# Autodesk Inventor assembly: assembly_hoop
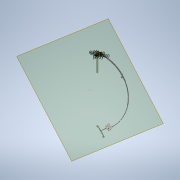
[picture p0: Inventor's stored thumbnail of the model, 180x180]
Saved by Autodesk Inventor 2021 (Build 250183000, 183)
## iProperties
Created: 2021-05-25
Part Number: assembly_hoop
Document SubType Name: Assembly
Designer: Watchdog
Mass: 37174 g
Surface Area: 24428.2 cm^2
Volume: 6220.71 cm^3
Density: 5.97585 g/cm^3
Author: Watchdog
## Documents named in this file (7)
- C:\Users\ocon0143\OneDrive - Flinders\Advn Mech Design Shared\6_Development\2_Design\inventor\assembly_hoop.iam
- C:\Users\ocon0143\OneDrive - Flinders\Advn Mech Design Shared\6_Development\2_Design\inventor\support\support_frameAssembly.iam
- C:\Users\ocon0143\OneDrive - Flinders\Advn Mech Design Shared\6_Development\2_Design\inventor\hoop_slider\hoops_sml_med_lrg.iam
- C:\Users\ocon0143\OneDrive - Flinders\Advn Mech Design Shared\6_Development\2_Design\inventor\support\reel\reelTab.ipt
- C:\Users\ocon0143\OneDrive - Flinders\Advn Mech Design Shared\6_Development\2_Design\inventor\support\reel\SKF_608.iam
- C:\Users\ocon0143\OneDrive - Flinders\Advn Mech Design Shared\6_Development\2_Design\inventor\support\reel\motorAssembly.iam
- C:\Users\ocon0143\OneDrive - Flinders\Advn Mech Design Shared\6_Development\2_Design\inventor\securing_mechanism\securingMechanism_variant_vertical_x\sm_varx.iam
## Components (6 placed, 6 different names)
1. support_frameAssembly:1 [sub-assembly] — Flush:1, Flush:2, Mate:1, Mate:6, Mate:10, Mate:11, Mate:12, Flush:4, Mate:20
2. hoops_sml_med_lrg:1 [sub-assembly] — Mate:6, Flush:4, Mate:19, Mate:20, Mate:21, Mate:22
3. reelTab:1 — Mate:10, Mate:11, Mate:12, Mate:13, Flush:3
4. SKF_608:1 [sub-assembly] — Mate:13, Flush:3, Mate:17, Mate:18
5. motorAssembly:1 [sub-assembly] — Mate:17, Mate:18
6. sm_varx:1 [sub-assembly] — Mate:19, Mate:21, Mate:22
## Relationships (16: Mate 12, Flush 4)
- Flush:1: support_frameAssembly:1
- Flush:2: support_frameAssembly:1
- Mate:1: support_frameAssembly:1
- Mate:6: support_frameAssembly:1 ↔ hoops_sml_med_lrg:1
- Mate:10: support_frameAssembly:1 ↔ reelTab:1
- Mate:11: support_frameAssembly:1 ↔ reelTab:1
- Mate:12: support_frameAssembly:1 ↔ reelTab:1
- Mate:13: reelTab:1 ↔ SKF_608:1
- Flush:3: reelTab:1 ↔ SKF_608:1
- Mate:17: SKF_608:1 ↔ motorAssembly:1
- Mate:18: SKF_608:1 ↔ motorAssembly:1
- Flush:4: support_frameAssembly:1 ↔ hoops_sml_med_lrg:1
- Mate:19: hoops_sml_med_lrg:1 ↔ sm_varx:1
- Mate:20: support_frameAssembly:1 ↔ hoops_sml_med_lrg:1
- Mate:21: hoops_sml_med_lrg:1 ↔ sm_varx:1
- Mate:22: hoops_sml_med_lrg:1 ↔ sm_varx:1
